# Autodesk Inventor assembly: ASY NDM 11.050 перегородка рама 2 вертикал
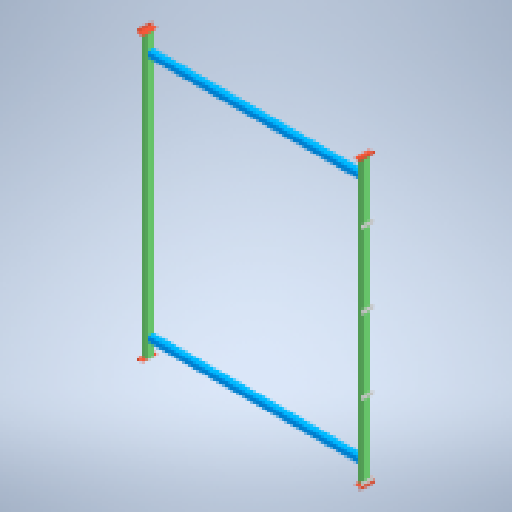
[picture p0: Inventor's stored thumbnail of the model, 512x512]
Saved by Autodesk Inventor 2025 (Build 290162010, 162A)
## iProperties
Created: 2024-08-12
Part Number: ASY NDM 11.050 перегородка рама 2 вертикал
Document SubType Name: Assembly
Designer: admin
_SolveAssemblyDoc: Frame Generator Solve Assembly
_Version: 25.0.0
Author: admin
## Documents named in this file (5)
- C:\Users\user\YandexDisk\домашниий пк\Inventor\Nadyim\CAD\Перегородка\ASY NDM 11.050 перегородка рама 2 вертикал.iam
- C:\Users\user\YandexDisk\домашниий пк\Inventor\Nadyim\CAD\Перегородка\NDM 11.042 рама 2 вертикал угол.ipt
- C:\Users\user\YandexDisk\домашниий пк\Inventor\Nadyim\CAD\Перегородка\ASY NDM 11.050 перегородка рама 2 вертикал\Frame\Frame 1723530770913.iam
- C:\Users\user\YandexDisk\домашниий пк\Inventor\Nadyim\CAD\кронштейн\NDM 4.0.9 кронштейн связь 9.ipt
- C:\Users\user\YandexDisk\домашниий пк\Inventor\Nadyim\CAD\кронштейн\NDM 11.028 кронштейн 28.ipt
## Components (10 placed, 4 different names)
1. NDM 11.042 рама 2 вертикал угол:1 — Mate:1, Mate:2, Flush:1
2. Frame 1723530770913:1 [sub-assembly] — Rigid:1, Rigid:2, Rigid:3, Rigid:4, Rigid:5
3. NDM 4.0.9 кронштейн связь 9:1 — Rigid:1
4. NDM 4.0.9 кронштейн связь 9:2 — Rigid:2
5. NDM 4.0.9 кронштейн связь 9:3 — Rigid:3
6. NDM 4.0.9 кронштейн связь 9:4 — Rigid:4
7. NDM 11.028 кронштейн 28:1 — Rigid:5
8. NDM 11.028 кронштейн 28:2
9. NDM 11.028 кронштейн 28:3
10. NDM 11.028 кронштейн 28:4
## Component patterns: (4 elements, first: NDM 11.028 кронштейн 28:1)
## Relationships (8: WeldJoint 5, Mate 2, Flush 1)
- Mate:1: NDM 11.042 рама 2 вертикал угол:1
- Mate:2: NDM 11.042 рама 2 вертикал угол:1
- Flush:1: NDM 11.042 рама 2 вертикал угол:1
- Rigid:1 [WeldJoint]: Frame 1723530770913:1 ↔ NDM 4.0.9 кронштейн связь 9:1
- Rigid:2 [WeldJoint]: Frame 1723530770913:1 ↔ NDM 4.0.9 кронштейн связь 9:2
- Rigid:3 [WeldJoint]: Frame 1723530770913:1 ↔ NDM 4.0.9 кронштейн связь 9:3
- Rigid:4 [WeldJoint]: Frame 1723530770913:1 ↔ NDM 4.0.9 кронштейн связь 9:4
- Rigid:5 [WeldJoint]: Frame 1723530770913:1 ↔ NDM 11.028 кронштейн 28:1
